# Autodesk Inventor assembly: UPPER_LEG_ASM
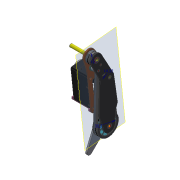
[picture p0: Inventor's stored thumbnail of the model, 180x180]
Saved by Autodesk Inventor 2019.4 (Build 234330000, 330)
## iProperties
Created: 2019-11-12
Part Number: UPPER_LEG_ASM
Material: 一般
Document SubType Name: Assembly
Designer: y6tada
Author: y6tada
## Documents named in this file (13)
- C:\Workspace\Yuni9\Inventor\Asm\UPPER_LEG\UPPER_LEG_ASM.iam
- C:\Workspace\Yuni9\Inventor\Libs\DYNAMIXEL\XM540\XM540_NO_BACK.iam
- C:\Workspace\Yuni9\Inventor\Asm\UPPER_LEG\ANKLE_DRIVER_LOD.ipt
- C:\Workspace\Yuni9\Inventor\Asm\UPPER_LEG\BELT_SUPPORT_INNER.iam
- C:\Workspace\Yuni9\Inventor\Asm\UPPER_LEG\KNEE_DRIVER_ASM.iam
- C:\Workspace\Yuni9\Inventor\Asm\UPPER_LEG\UPPER_LEG_OUTER_FRAME.ipt
- C:\Workspace\Yuni9\Inventor\Asm\UPPER_LEG\COXA_PITCH_DRIVER_PULLEY.iam
- C:\Workspace\Yuni9\Inventor\Asm\UPPER_LEG\SERVO_MOUNT_TIP.ipt
- C:\Workspace\Yuni9\Inventor\Asm\UPPER_LEG\SERVO_BOTTOM_SPACER.ipt
- C:\Workspace\Yuni9\Inventor\Asm\UPPER_LEG\UPPER_LEG_MIDDLE_FRAME.ipt
- C:\Workspace\Yuni9\Inventor\Asm\UPPER_LEG\BELT_TENSIONER_ASM.iam
- C:\Workspace\Yuni9\Inventor\Asm\UPPER_LEG\OUTER_COVER.ipt
- C:\Workspace\Yuni9\Inventor\Asm\UPPER_LEG\UPPER_LEG_ASM\デザイン アクセラレータ\歯付きベルト伝達2.iam
## Components (12 placed, 12 different names)
1. UPPER_LEG_OUTER_FRAME:1 — フラッシュ:4, メイト:39, メイト:51, フラッシュ:6, フラッシュ:7, メイト:52, フラッシュ:8, フラッシュ:9, 対称度:1
2. XM540_NO_BACK:1 [sub-assembly] — メイト:36, メイト:37, メイト:38, メイト:40, メイト:41, メイト:42, フラッシュ:5, メイト:47
3. ANKLE_DRIVER_LOD:1 — メイト:3
4. BELT_SUPPORT_INNER:1 [sub-assembly] — メイト:51, フラッシュ:6
5. KNEE_DRIVER_ASM:1 [sub-assembly] — フラッシュ:7, メイト:52
6. COXA_PITCH_DRIVER_PULLEY:1 [sub-assembly] — フラッシュ:8
7. SERVO_MOUNT_TIP:1 — メイト:36, メイト:37, メイト:38, メイト:39
8. SERVO_BOTTOM_SPACER:1 — メイト:40, メイト:41, メイト:42, メイト:45
9. UPPER_LEG_MIDDLE_FRAME:1 — メイト:45, 対称度:1
10. BELT_TENSIONER_ASM:1 [sub-assembly]
11. OUTER_COVER:1 — フラッシュ:9, フラッシュ:10, フラッシュ:11
12. 歯付きベルト伝達:1 [sub-assembly]
## Relationships (29: Mate 19, Flush 8, Angle 1, Symmetry 1)
- [Mate]: COXA_PITCH_DRIVER_PULLEY:1
- メイト:3 [Mate]: ANKLE_DRIVER_LOD:1
- [Mate]: COXA_PITCH_DRIVER_PULLEY:1
- [Mate] (1 mm): ANKLE_DRIVER_LOD:1 ↔ COXA_PITCH_DRIVER_PULLEY:1
- フラッシュ:4 [Flush]: UPPER_LEG_OUTER_FRAME:1
- メイト:36 [Mate]: XM540_NO_BACK:1 ↔ SERVO_MOUNT_TIP:1
- メイト:37 [Mate]: XM540_NO_BACK:1 ↔ SERVO_MOUNT_TIP:1
- メイト:38 [Mate]: XM540_NO_BACK:1 ↔ SERVO_MOUNT_TIP:1
- メイト:39 [Mate]: UPPER_LEG_OUTER_FRAME:1 ↔ SERVO_MOUNT_TIP:1
- メイト:40 [Mate]: XM540_NO_BACK:1 ↔ SERVO_BOTTOM_SPACER:1
- メイト:41 [Mate]: XM540_NO_BACK:1 ↔ SERVO_BOTTOM_SPACER:1
- メイト:42 [Mate]: XM540_NO_BACK:1 ↔ SERVO_BOTTOM_SPACER:1
- メイト:45 [Mate]: SERVO_BOTTOM_SPACER:1 ↔ UPPER_LEG_MIDDLE_FRAME:1
- メイト:46 [Mate]
- 角度:1 [Angle] (6 deg)
- フラッシュ:5 [Flush] (75 mm): XM540_NO_BACK:1
- メイト:47 [Mate]: XM540_NO_BACK:1
- [Mate]: UPPER_LEG_OUTER_FRAME:1 ↔ BELT_TENSIONER_ASM:1
- [Mate] (0.1 mm): UPPER_LEG_OUTER_FRAME:1 ↔ BELT_TENSIONER_ASM:1
- [Mate]: UPPER_LEG_OUTER_FRAME:1 ↔ BELT_TENSIONER_ASM:1
- メイト:51 [Mate]: UPPER_LEG_OUTER_FRAME:1 ↔ BELT_SUPPORT_INNER:1
- フラッシュ:6 [Flush]: UPPER_LEG_OUTER_FRAME:1 ↔ BELT_SUPPORT_INNER:1
- フラッシュ:7 [Flush]: UPPER_LEG_OUTER_FRAME:1 ↔ KNEE_DRIVER_ASM:1
- メイト:52 [Mate]: UPPER_LEG_OUTER_FRAME:1 ↔ KNEE_DRIVER_ASM:1
- フラッシュ:8 [Flush]: UPPER_LEG_OUTER_FRAME:1 ↔ COXA_PITCH_DRIVER_PULLEY:1
- フラッシュ:9 [Flush]: UPPER_LEG_OUTER_FRAME:1 ↔ OUTER_COVER:1
- フラッシュ:10 [Flush]: OUTER_COVER:1
- フラッシュ:11 [Flush]: OUTER_COVER:1
- 対称度:1 [Symmetry]: UPPER_LEG_OUTER_FRAME:1 ↔ UPPER_LEG_MIDDLE_FRAME:1
